# Autodesk Inventor assembly: электроника
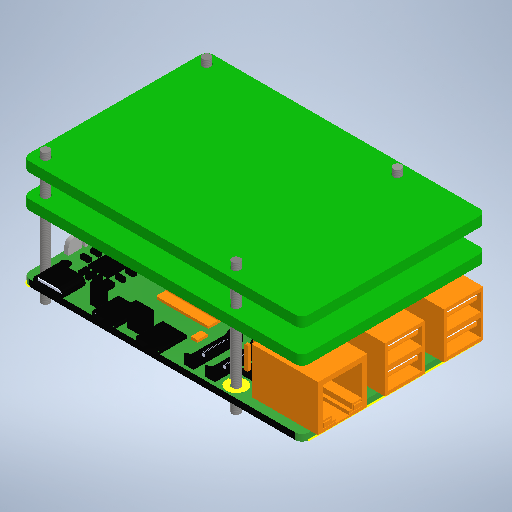
[picture p0: Inventor's stored thumbnail of the model, 512x512]
Saved by Autodesk Inventor 2025 (Build 290162000, 162)
## iProperties
Created: 2025-02-25
Part Number: электроника
Document SubType Name: Assembly
Designer: volko
Author: volko
## Documents named in this file (4)
- C:\Users\volko\Desktop\диплом\Модели\детали\электроника.iam
- C:\Users\volko\Desktop\диплом\Модели\детали\Raspberry Pi 5.ipt
- C:\Users\volko\Desktop\диплом\Модели\детали\плата двигателей.ipt
- C:\Users\volko\Desktop\диплом\Модели\детали\стандартные изделия\ru-RU\DIN 976-1 A\DIN 976-1 - M2,5 x 40 - A.ipt
## Components (7 placed, 3 different names)
1. Raspberry Pi 5:1 — Заподлицо:1, Заподлицо:2, Заподлицо:3, Совмещение:1, Совмещение:2, Совмещение:3, Совмещение:4, Совмещение:5, Заподлицо:10, Заподлицо:11, Заподлицо:12
2. плата двигателей:1 — Заподлицо:4, Заподлицо:5, Заподлицо:8
3. плата двигателей:2 — Заподлицо:6, Заподлицо:7, Заподлицо:9
4. DIN 976-1 A M2,5 x 40:2 — Совмещение:2, Заподлицо:12
5. DIN 976-1 A M2,5 x 40:3 — Совмещение:1, Заподлицо:11
6. DIN 976-1 A M2,5 x 40:4 — Совмещение:4, Заподлицо:10
7. DIN 976-1 A M2,5 x 40:5 — Совмещение:3, Совмещение:5
## Relationships (17: Flush 12, Mate 5)
- Заподлицо:1 [Flush]: Raspberry Pi 5:1
- Заподлицо:2 [Flush]: Raspberry Pi 5:1
- Заподлицо:3 [Flush]: Raspberry Pi 5:1
- Заподлицо:4 [Flush]: плата двигателей:1
- Заподлицо:5 [Flush]: плата двигателей:1
- Заподлицо:6 [Flush]: плата двигателей:2
- Заподлицо:7 [Flush]: плата двигателей:2
- Заподлицо:8 [Flush] (20 mm): плата двигателей:1
- Заподлицо:9 [Flush] (30 mm): плата двигателей:2
- Совмещение:1 [Mate]: Raspberry Pi 5:1 ↔ DIN 976-1 A M2,5 x 40:3
- Совмещение:2 [Mate]: Raspberry Pi 5:1 ↔ DIN 976-1 A M2,5 x 40:2
- Совмещение:3 [Mate]: Raspberry Pi 5:1 ↔ DIN 976-1 A M2,5 x 40:5
- Совмещение:4 [Mate]: Raspberry Pi 5:1 ↔ DIN 976-1 A M2,5 x 40:4
- Совмещение:5 [Mate] (5 mm): Raspberry Pi 5:1 ↔ DIN 976-1 A M2,5 x 40:5
- Заподлицо:10 [Flush] (5 mm): Raspberry Pi 5:1 ↔ DIN 976-1 A M2,5 x 40:4
- Заподлицо:11 [Flush] (5 mm): Raspberry Pi 5:1 ↔ DIN 976-1 A M2,5 x 40:3
- Заподлицо:12 [Flush] (5 mm): Raspberry Pi 5:1 ↔ DIN 976-1 A M2,5 x 40:2
